# Autodesk Inventor assembly: Zespół1
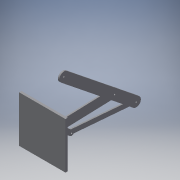
[picture p0: Inventor's stored thumbnail of the model, 180x180]
Saved by Autodesk Inventor 2017 (Build 210142000, 142)
## iProperties
Part Number: Zespół1
Material: Ogólny
Document SubType Name: Assembly
Designer: Damian
Author: Damian
## Documents named in this file (6)
- C:\Users\Damian\Documents\Inventor\Nowe\Zespół1.iam
- C:\Users\Damian\Documents\Inventor\Nowe\segment1.ipt
- C:\Users\Damian\Documents\Inventor\Nowe\segment2.ipt
- C:\Users\Damian\Documents\Inventor\Nowe\korba.ipt
- C:\Users\Damian\Documents\Inventor\Nowe\korbowód.ipt
- C:\Users\Damian\Documents\Inventor\Nowe\podstawa.ipt
## Components (5 placed, 5 different names)
1. segment1:1 — Wstaw:1, Wstaw:2, Wstaw:5
2. segment2:1 — Wstaw:1, Wstaw:4
3. korbowód:1 — Wstaw:3, Wstaw:4
4. korba:1 — Wstaw:2, Wstaw:3
5. podstawa:1 — Wstaw:5
## Relationships (5: Insert 5)
- Wstaw:1 [Insert]: segment1:1 ↔ segment2:1
- Wstaw:2 [Insert]: segment1:1 ↔ korba:1
- Wstaw:3 [Insert]: korbowód:1 ↔ korba:1
- Wstaw:4 [Insert]: segment2:1 ↔ korbowód:1
- Wstaw:5 [Insert]: segment1:1 ↔ podstawa:1
